# Autodesk Inventor assembly: ShortElevatorFrame
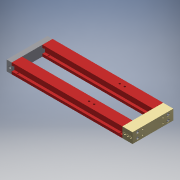
[picture p0: Inventor's stored thumbnail of the model, 180x180]
Saved by Autodesk Inventor 2019 (Build 230136000, 136)
## iProperties
Created: 2019-09-28
Part Number: ShortElevatorFrame
Document SubType Name: Assembly
Designer: james
Author: james
## Documents named in this file (4)
- F:\JimsDesign\Jims2020FTC\ShortElevatorFrame.iam
- F:\JimsDesign\Jims2020FTC\ElvatorEnd.iam
- F:\JimsDesign\Jims2020FTC\ElvatorBottom.iam
- F:\JimsDesign\Jims2020FTC\ShortBeamSplit.ipt
## Components (4 placed, 3 different names)
1. ElvatorBottom:1 [sub-assembly] — Mate:7, Mate:8, Mate:9
2. ElvatorEnd:2 [sub-assembly] — Mate:1, Mate:2, Mate:3, Mate:4, Mate:5, Mate:6
3. ShortBeamSplit:1 — Mate:2, Mate:4, Mate:5, Mate:8
4. ShortBeamSplit:2 — Mate:1, Mate:3, Mate:6, Mate:7, Mate:9
## Relationships (9: Mate 9)
- Mate:1: ElvatorEnd:2 ↔ ShortBeamSplit:2
- Mate:2: ElvatorEnd:2 ↔ ShortBeamSplit:1
- Mate:3: ElvatorEnd:2 ↔ ShortBeamSplit:2
- Mate:4: ElvatorEnd:2 ↔ ShortBeamSplit:1
- Mate:5: ElvatorEnd:2 ↔ ShortBeamSplit:1
- Mate:6: ElvatorEnd:2 ↔ ShortBeamSplit:2
- Mate:7: ElvatorBottom:1 ↔ ShortBeamSplit:2
- Mate:8: ElvatorBottom:1 ↔ ShortBeamSplit:1
- Mate:9: ElvatorBottom:1 ↔ ShortBeamSplit:2
